# Autodesk Inventor assembly: erp42
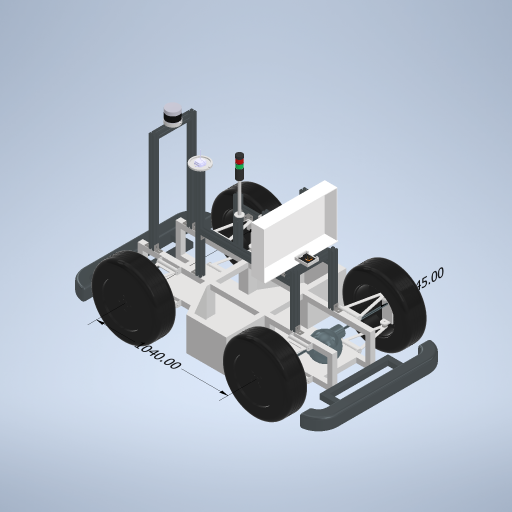
[picture p0: Inventor's stored thumbnail of the model, 512x512]
Saved by Autodesk Inventor 2023 (Build 270158000, 158)
## iProperties
Created: 2024-02-06
Part Number: erp42
Document SubType Name: Assembly
Designer: ps737
Author: ps737
## Documents named in this file (29)
- C:\Users\ps737\OneDrive\바탕 화면\2024 ERP42\erp42.iam
- C:\Users\ps737\OneDrive\바탕 화면\2024 ERP42\body.ipt
- C:\Users\ps737\OneDrive\바탕 화면\2024 ERP42\bumper.ipt
- C:\Users\ps737\OneDrive\바탕 화면\2024 ERP42\body_braket.ipt
- C:\Users\ps737\OneDrive\바탕 화면\2024 ERP42\link.ipt
- C:\Users\ps737\OneDrive\바탕 화면\2024 ERP42\wheel.ipt
- C:\Users\ps737\OneDrive\바탕 화면\2024 ERP42\wheel_bolt.ipt
- C:\Users\ps737\OneDrive\바탕 화면\2024 ERP42\프로파일\34.ipt
- C:\Users\ps737\OneDrive\바탕 화면\2024 ERP42\프로파일\76.ipt
- C:\Users\ps737\OneDrive\바탕 화면\2024 ERP42\프로파일\79.ipt
- C:\Users\ps737\OneDrive\바탕 화면\2024 ERP42\프로파일\26.ipt
- C:\Users\ps737\OneDrive\바탕 화면\2024 ERP42\프로파일\71.ipt
- C:\Users\ps737\OneDrive\바탕 화면\2024 ERP42\lidar_case.ipt
- C:\Users\ps737\OneDrive\바탕 화면\2024 ERP42\86-0138 REV 2, ENVELOPE, VLP-32C M12M.iam
- C:\Users\ps737\OneDrive\바탕 화면\2024 ERP42\gps_case.ipt
- C:\Users\ps737\OneDrive\바탕 화면\2024 ERP42\UBLOX_ANN-MB-00_GNSS_ANTENNA.ipt
- C:\Users\ps737\OneDrive\바탕 화면\2024 ERP42\프로파일\40.5.ipt
- C:\Users\ps737\OneDrive\바탕 화면\2024 ERP42\imu_case.ipt
- C:\Users\ps737\OneDrive\바탕 화면\2024 ERP42\MTi 600-series STEP files\MTi-600 DEV assembly.iam
- C:\Users\ps737\OneDrive\바탕 화면\2024 ERP42\L자 브라켓.ipt
- C:\Users\ps737\OneDrive\바탕 화면\2024 ERP42\wheel_braket_13.ipt
- C:\Users\ps737\OneDrive\바탕 화면\2024 ERP42\wheel_braket_24.ipt
- C:\Users\ps737\OneDrive\바탕 화면\2024 ERP42\base_link.ipt
- base_link.ipt
- C:\Users\ps737\OneDrive\바탕 화면\2024 ERP42\gps_case_2.ipt
- C:\Users\ps737\OneDrive\바탕 화면\2024 ERP42\프로파일\8.ipt
- C:\Users\ps737\OneDrive\바탕 화면\2024 ERP42\프로파일\36.ipt
- C:\Users\ps737\OneDrive\바탕 화면\2024 ERP42\monitor_case.ipt
- C:\Users\ps737\OneDrive\바탕 화면\2024 ERP42\led.ipt
## Components (74 placed, 27 different names)
1. body:1 — 메이트:1, 메이트:2, 메이트:3, 메이트:4, 메이트:5, 메이트:6, 메이트:9, 메이트:12, 메이트:60, 메이트:61, 플러쉬:1, 플러쉬:3, 플러쉬:4, 메이트:62, 메이트:64, 메이트:65, 플러쉬:6, 플러쉬:7, 플러쉬:8, 메이트:77, 메이트:78, 메이트:79, 플러쉬:9, 플러쉬:10, 플러쉬:11, 메이트:86, 메이트:89, 플러쉬:16, 메이트:90, 메이트:91, 플러쉬:17, 플러쉬:18, 메이트:107, 메이트:108, 플러쉬:21, 플러쉬:22, 메이트:109, 메이트:110, 메이트:124, 플러쉬:28, 각도:18, 플러쉬:29, 각도:19, 플러쉬:31, 플러쉬:32, 플러쉬:33, 메이트:152, 메이트:153, 메이트:154, 각도:20, 각도:21, 각도:22, 각도:23, 메이트:192, 플러쉬:34, 메이트:194, 플러쉬:35, 메이트:196, 플러쉬:36, 메이트:198, 플러쉬:37, 메이트:200, 플러쉬:38, 메이트:202, 플러쉬:39, 메이트:204, 메이트:206, 플러쉬:41, 메이트:209, 플러쉬:42, 메이트:241, 메이트:242
2. bumper:1 — 메이트:1, 메이트:2, 플러쉬:6, 플러쉬:10
3. bumper:2 — 메이트:3, 메이트:4, 플러쉬:7, 플러쉬:11, 플러쉬:58
4. body_braket:5 — 메이트:5, 플러쉬:32, 메이트:145, 메이트:151, 메이트:153
5. body_braket:7 — 메이트:6, 메이트:133, 메이트:134, 플러쉬:29, 플러쉬:30
6. body_braket:10 — 메이트:9, 플러쉬:3, 메이트:65, 메이트:144, 메이트:150
7. body_braket:12 — 메이트:12, 플러쉬:1, 메이트:62, 메이트:135, 메이트:136, 플러쉬:30, 플러쉬:40
8. body_braket:15 — 메이트:61, 메이트:140, 메이트:143, 플러쉬:31, 메이트:154
9. body_braket:16 — 메이트:60, 플러쉬:4, 메이트:64, 메이트:141, 메이트:142
10. body_braket:17 — 메이트:79, 플러쉬:33, 메이트:146, 메이트:148, 메이트:152
11. body_braket:18 — 메이트:77, 메이트:78, 플러쉬:9, 메이트:147, 메이트:149
12. 76:1 — 메이트:86, 메이트:89, 플러쉬:16, 메이트:105, 메이트:106, 각도:15, 각도:16, 메이트:207, 메이트:229, 플러쉬:54, 메이트:233
13. 79:1 — 메이트:90, 플러쉬:18, 메이트:94, 플러쉬:19, 플러쉬:20, 메이트:122, 메이트:193, 메이트:195
14. 79:2 — 메이트:91, 플러쉬:17, 메이트:123, 메이트:197, 메이트:199
15. 26:1 — 메이트:94, 플러쉬:19, 플러쉬:20, 메이트:101, 각도:13, 메이트:102
16. lidar_case:1 — 메이트:99, 메이트:100, 각도:12, 메이트:101
17. 86-0138 REV 2, ENVELOPE, VLP-32C M12M:1 [sub-assembly] — 메이트:99, 메이트:100, 각도:12, 각도:13, 메이트:102
18. gps_case:1 — 메이트:103, 각도:14, 메이트:104, 메이트:105, 메이트:106, 각도:16
19. UBLOX_ANN-MB-00_GNSS_ANTENNA:1 — 메이트:103, 각도:14, 메이트:104, 각도:15
20. 40.5:1 — 메이트:107, 플러쉬:21, 메이트:109, 메이트:111, 플러쉬:23, 플러쉬:24, 플러쉬:25, 메이트:201, 메이트:225, 플러쉬:52, 플러쉬:59
21. 40.5:2 — 메이트:108, 플러쉬:22, 메이트:110, 메이트:112, 메이트:114, 플러쉬:26, 메이트:205, 플러쉬:42, 메이트:224, 플러쉬:51
22. 34:1 — 메이트:111, 플러쉬:23, 플러쉬:24, 메이트:113, 메이트:115, 메이트:119, 메이트:120, 각도:17, 메이트:122, 메이트:123, 메이트:220, 메이트:222
23. 71:1 — 메이트:112, 메이트:113, 플러쉬:25, 메이트:211, 메이트:221, 플러쉬:48, 메이트:226, 메이트:230, 메이트:231, 플러쉬:55, 메이트:235, 플러쉬:57
24. 71:2 — 메이트:114, 플러쉬:26, 메이트:115, 메이트:125, 플러쉬:43, 메이트:213, 플러쉬:44, 메이트:215, 메이트:216, 플러쉬:46, 메이트:219, 플러쉬:49, 플러쉬:50, 메이트:223, 메이트:228, 메이트:232, 플러쉬:56
25. imu_case:1 — 메이트:116, 메이트:117, 메이트:118, 메이트:119, 메이트:120, 각도:17
26. MTi-600 DEV assembly:1 [sub-assembly] — 메이트:116, 메이트:117, 메이트:118
27. 40.5:3 — 메이트:124, 플러쉬:28, 메이트:125, 메이트:203, 메이트:212, 메이트:214, 메이트:227, 플러쉬:53, 메이트:234
28. link:19 — 메이트:129, 메이트:130, 메이트:133, 메이트:134
29. wheel_braket_13:1 — 메이트:131, 메이트:132, 각도:19, 메이트:137, 메이트:139, 메이트:179, 각도:23, 메이트:185
30. wheel_bolt:11 — 메이트:129, 메이트:130, 메이트:131, 메이트:132
31. link:20 — 메이트:135, 메이트:136, 각도:18, 메이트:138, 메이트:240
32. wheel_bolt:12 — 메이트:137, 메이트:138, 메이트:139, 메이트:240
33. link:21 — 메이트:141, 메이트:142, 메이트:175, 메이트:177
34. link:22 — 메이트:140, 메이트:143, 메이트:176, 메이트:178, 메이트:184
35. link:23 — 메이트:146, 메이트:148, 메이트:172, 메이트:174
36. link:24 — 메이트:147, 메이트:149, 메이트:171, 메이트:173
37. link:25 — 메이트:144, 메이트:150, 메이트:167, 메이트:168
38. link:26 — 메이트:145, 메이트:151, 메이트:169, 메이트:170
39. wheel:1 — 메이트:186, 메이트:187
40. wheel:2 — 메이트:179, 메이트:185
41. wheel:3 — 메이트:190, 메이트:191
42. wheel:4 — 메이트:188, 메이트:189, 메이트:208, 메이트:210
43. wheel_braket_13:2 — 메이트:155, 메이트:156, 메이트:161, 메이트:162, 각도:21, 메이트:190, 메이트:191
44. wheel_braket_24:1 — 메이트:180, 메이트:181, 메이트:182, 메이트:183, 각도:20, 메이트:186, 메이트:187
45. wheel_braket_24:2 — 메이트:157, 메이트:158, 메이트:163, 메이트:164, 각도:22, 메이트:188, 메이트:189
46. wheel_bolt:13 — 메이트:158, 메이트:163, 메이트:172, 메이트:174
47. wheel_bolt:14 — 메이트:155, 메이트:161, 메이트:169, 메이트:170
48. wheel_bolt:15 — 메이트:157, 메이트:164, 메이트:171, 메이트:173
49. wheel_bolt:16 — 메이트:156, 메이트:162, 메이트:167, 메이트:168
50. wheel_bolt:17 — 메이트:175, 메이트:177, 메이트:180, 메이트:181, 메이트:183
51. wheel_bolt:18 — 메이트:176, 메이트:178, 메이트:182, 메이트:184
52. L자 브라켓:1 — 메이트:194, 메이트:195, 플러쉬:35
53. L자 브라켓:2 — 메이트:192, 메이트:193, 플러쉬:34
54. L자 브라켓:3 — 메이트:196, 메이트:197, 플러쉬:36
55. L자 브라켓:4 — 메이트:198, 메이트:199, 플러쉬:37
56. L자 브라켓:5 — 메이트:202, 메이트:203, 플러쉬:39
57. L자 브라켓:6 — 메이트:200, 메이트:201, 플러쉬:38, 플러쉬:59
58. L자 브라켓:7 — 메이트:204, 메이트:205, 플러쉬:40
59. L자 브라켓:8 — 메이트:206, 메이트:207, 플러쉬:41
60. base_link:1 — 메이트:208, 메이트:209, 메이트:210
61. gps_case_2:1 — 메이트:211, 메이트:212, 플러쉬:43
62. 8:1 — 메이트:213, 플러쉬:44, 메이트:214, 메이트:217, 메이트:218, 메이트:237, 메이트:238, 메이트:239
63. L자 브라켓:9 — 메이트:215, 플러쉬:46, 메이트:217
64. L자 브라켓:10 — 메이트:216, 메이트:218, 플러쉬:50
65. L자 브라켓:11 — 메이트:219, 메이트:220, 플러쉬:49
66. L자 브라켓:12 — 메이트:221, 메이트:222, 플러쉬:48
67. L자 브라켓:13 — 메이트:229, 메이트:230, 플러쉬:54
68. L자 브라켓:14 — 메이트:223, 메이트:224, 플러쉬:51
69. L자 브라켓:15 — 메이트:225, 메이트:226, 플러쉬:52
70. L자 브라켓:17 — 메이트:227, 메이트:228, 플러쉬:53
71. 36:1 — 메이트:231, 플러쉬:55, 메이트:233, 메이트:236
72. 36:2 — 메이트:232, 플러쉬:56, 메이트:234
73. monitor_case:1 — 메이트:235, 메이트:236, 플러쉬:57
74. led:1 — 메이트:237, 메이트:238, 메이트:239
## Relationships (219: Mate 157, Flush 50, Angle 12)
- 메이트:1 [Mate]: body:1 ↔ bumper:1
- 메이트:2 [Mate]: body:1 ↔ bumper:1
- 메이트:3 [Mate]: body:1 ↔ bumper:2
- 메이트:4 [Mate]: body:1 ↔ bumper:2
- 메이트:5 [Mate]: body:1 ↔ body_braket:5
- 메이트:6 [Mate]: body:1 ↔ body_braket:7
- 메이트:9 [Mate]: body:1 ↔ body_braket:10
- 메이트:12 [Mate]: body:1 ↔ body_braket:12
- 메이트:60 [Mate]: body:1 ↔ body_braket:16
- 메이트:61 [Mate]: body:1 ↔ body_braket:15
- 플러쉬:1 [Flush]: body:1 ↔ body_braket:12
- 플러쉬:3 [Flush]: body:1 ↔ body_braket:10
- 플러쉬:4 [Flush]: body:1 ↔ body_braket:16
- 메이트:62 [Mate] (230 mm): body:1 ↔ body_braket:12
- 메이트:64 [Mate] (190 mm): body:1 ↔ body_braket:16
- 메이트:65 [Mate] (190 mm): body:1 ↔ body_braket:10
- 플러쉬:6 [Flush] (-25 mm): body:1 ↔ bumper:1
- 플러쉬:7 [Flush] (-25 mm): body:1 ↔ bumper:2
- 플러쉬:8 [Flush] (105 mm): body:1
- 메이트:77 [Mate]: body:1 ↔ body_braket:18
- 메이트:78 [Mate] (230 mm): body:1 ↔ body_braket:18
- 메이트:79 [Mate]: body:1 ↔ body_braket:17
- 플러쉬:9 [Flush]: body:1 ↔ body_braket:18
- 플러쉬:10 [Flush] (100 mm): body:1 ↔ bumper:1
- 플러쉬:11 [Flush] (100 mm): body:1 ↔ bumper:2
- 메이트:86 [Mate]: body:1 ↔ 76:1
- 메이트:89 [Mate] (40 mm): body:1 ↔ 76:1
- 플러쉬:16 [Flush]: body:1 ↔ 76:1
- 메이트:90 [Mate]: body:1 ↔ 79:1
- 메이트:91 [Mate]: body:1 ↔ 79:2
- 플러쉬:17 [Flush]: body:1 ↔ 79:2
- 플러쉬:18 [Flush]: body:1 ↔ 79:1
- 메이트:94 [Mate]: 79:1 ↔ 26:1
- 플러쉬:19 [Flush]: 79:1 ↔ 26:1
- 플러쉬:20 [Flush]: 79:1 ↔ 26:1
- 메이트:99 [Mate]: lidar_case:1 ↔ 86-0138 REV 2, ENVELOPE, VLP-32C M12M:1
- 메이트:100 [Mate]: lidar_case:1 ↔ 86-0138 REV 2, ENVELOPE, VLP-32C M12M:1
- 각도:12 [Angle] (270 deg): lidar_case:1 ↔ 86-0138 REV 2, ENVELOPE, VLP-32C M12M:1
- 메이트:101 [Mate]: 26:1 ↔ lidar_case:1
- 각도:13 [Angle] (0 deg): 26:1 ↔ 86-0138 REV 2, ENVELOPE, VLP-32C M12M:1
- 메이트:102 [Mate]: 26:1 ↔ 86-0138 REV 2, ENVELOPE, VLP-32C M12M:1
- 메이트:103 [Mate]: gps_case:1 ↔ UBLOX_ANN-MB-00_GNSS_ANTENNA:1
- 각도:14 [Angle] (270 deg): gps_case:1 ↔ UBLOX_ANN-MB-00_GNSS_ANTENNA:1
- 메이트:104 [Mate]: gps_case:1 ↔ UBLOX_ANN-MB-00_GNSS_ANTENNA:1
- 메이트:105 [Mate]: 76:1 ↔ gps_case:1
- 메이트:106 [Mate]: 76:1 ↔ gps_case:1
- 각도:15 [Angle] (0 deg): 76:1 ↔ UBLOX_ANN-MB-00_GNSS_ANTENNA:1
- 각도:16 [Angle] (270 deg): 76:1 ↔ gps_case:1
- 메이트:107 [Mate]: body:1 ↔ 40.5:1
- 메이트:108 [Mate]: body:1 ↔ 40.5:2
- 플러쉬:21 [Flush]: body:1 ↔ 40.5:1
- 플러쉬:22 [Flush]: body:1 ↔ 40.5:2
- 메이트:109 [Mate] (200 mm): body:1 ↔ 40.5:1
- 메이트:110 [Mate] (200 mm): body:1 ↔ 40.5:2
- 메이트:111 [Mate]: 40.5:1 ↔ 34:1
- 플러쉬:23 [Flush]: 40.5:1 ↔ 34:1
- 플러쉬:24 [Flush] (28 mm): 40.5:1 ↔ 34:1
- 메이트:112 [Mate]: 40.5:2 ↔ 71:1
- 메이트:113 [Mate]: 34:1 ↔ 71:1
- 플러쉬:25 [Flush]: 40.5:1 ↔ 71:1
- 메이트:114 [Mate]: 40.5:2 ↔ 71:2
- 플러쉬:26 [Flush]: 40.5:2 ↔ 71:2
- 메이트:115 [Mate]: 34:1 ↔ 71:2
- 메이트:116 [Mate]: imu_case:1 ↔ MTi-600 DEV assembly:1
- 메이트:117 [Mate]: imu_case:1 ↔ MTi-600 DEV assembly:1
- 메이트:118 [Mate]: imu_case:1 ↔ MTi-600 DEV assembly:1
- 메이트:119 [Mate]: 34:1 ↔ imu_case:1
- 메이트:120 [Mate]: 34:1 ↔ imu_case:1
- 각도:17 [Angle] (0 deg): 34:1 ↔ imu_case:1
- 메이트:122 [Mate] (1038 mm): 79:1 ↔ 34:1
- 메이트:123 [Mate] (1038 mm): 79:2 ↔ 34:1
- 메이트:124 [Mate]: body:1 ↔ 40.5:3
- 플러쉬:28 [Flush]: body:1 ↔ 40.5:3
- 메이트:125 [Mate]: 71:2 ↔ 40.5:3
- 메이트:129 [Mate]: link:19 ↔ wheel_bolt:11
- 메이트:130 [Mate]: link:19 ↔ wheel_bolt:11
- 메이트:131 [Mate]: wheel_braket_13:1 ↔ wheel_bolt:11
- 메이트:132 [Mate]: wheel_braket_13:1 ↔ wheel_bolt:11
- 메이트:133 [Mate]: body_braket:7 ↔ link:19
- 메이트:134 [Mate]: body_braket:7 ↔ link:19
- 메이트:135 [Mate]: body_braket:12 ↔ link:20
- 메이트:136 [Mate]: body_braket:12 ↔ link:20
- 각도:18 [Angle] (0 deg): body:1 ↔ link:20
- 플러쉬:29 [Flush]: body:1 ↔ body_braket:7
- 각도:19 [Angle] (180 deg): body:1 ↔ wheel_braket_13:1
- 플러쉬:30 [Flush]: body_braket:7 ↔ body_braket:12
- 메이트:137 [Mate]: wheel_braket_13:1 ↔ wheel_bolt:12
- 메이트:138 [Mate]: link:20 ↔ wheel_bolt:12
- 메이트:139 [Mate]: wheel_braket_13:1 ↔ wheel_bolt:12
- 메이트:140 [Mate]: body_braket:15 ↔ link:22
- 메이트:141 [Mate]: body_braket:16 ↔ link:21
- 메이트:142 [Mate]: body_braket:16 ↔ link:21
- 메이트:143 [Mate]: body_braket:15 ↔ link:22
- 플러쉬:31 [Flush]: body:1 ↔ body_braket:15
- 플러쉬:32 [Flush]: body:1 ↔ body_braket:5
- 플러쉬:33 [Flush]: body:1 ↔ body_braket:17
- 메이트:144 [Mate]: body_braket:10 ↔ link:25
- 메이트:145 [Mate]: body_braket:5 ↔ link:26
- 메이트:146 [Mate]: body_braket:17 ↔ link:23
- 메이트:147 [Mate]: body_braket:18 ↔ link:24
- 메이트:148 [Mate]: body_braket:17 ↔ link:23
- 메이트:149 [Mate]: body_braket:18 ↔ link:24
- 메이트:150 [Mate]: body_braket:10 ↔ link:25
- 메이트:151 [Mate]: body_braket:5 ↔ link:26
- 메이트:152 [Mate] (230 mm): body:1 ↔ body_braket:17
- 메이트:153 [Mate] (190 mm): body:1 ↔ body_braket:5
- 메이트:154 [Mate] (190 mm): body:1 ↔ body_braket:15
- 메이트:155 [Mate]: wheel_braket_13:2 ↔ wheel_bolt:14
- 메이트:156 [Mate]: wheel_braket_13:2 ↔ wheel_bolt:16
- 메이트:157 [Mate]: wheel_braket_24:2 ↔ wheel_bolt:15
- 메이트:158 [Mate]: wheel_braket_24:2 ↔ wheel_bolt:13
- 메이트:161 [Mate]: wheel_braket_13:2 ↔ wheel_bolt:14
- 메이트:162 [Mate]: wheel_braket_13:2 ↔ wheel_bolt:16
- 메이트:163 [Mate]: wheel_braket_24:2 ↔ wheel_bolt:13
- 메이트:164 [Mate]: wheel_braket_24:2 ↔ wheel_bolt:15
- 메이트:167 [Mate]: link:25 ↔ wheel_bolt:16
- 메이트:168 [Mate]: link:25 ↔ wheel_bolt:16
- 메이트:169 [Mate]: link:26 ↔ wheel_bolt:14
- 메이트:170 [Mate]: link:26 ↔ wheel_bolt:14
- 메이트:171 [Mate]: link:24 ↔ wheel_bolt:15
- 메이트:172 [Mate]: link:23 ↔ wheel_bolt:13
- 메이트:173 [Mate]: link:24 ↔ wheel_bolt:15
- 메이트:174 [Mate]: link:23 ↔ wheel_bolt:13
- 메이트:175 [Mate]: link:21 ↔ wheel_bolt:17
- 메이트:176 [Mate]: link:22 ↔ wheel_bolt:18
- 메이트:177 [Mate]: link:21 ↔ wheel_bolt:17
- 메이트:178 [Mate]: link:22 ↔ wheel_bolt:18
- 메이트:179 [Mate]: wheel_braket_13:1 ↔ wheel:2
- 메이트:180 [Mate]: wheel_braket_24:1 ↔ wheel_bolt:17
- 메이트:181 [Mate]: wheel_braket_24:1 ↔ wheel_bolt:17
- 메이트:182 [Mate]: wheel_braket_24:1 ↔ wheel_bolt:18
- 메이트:183 [Mate]: wheel_braket_24:1 ↔ wheel_bolt:17
- 메이트:184 [Mate]: link:22 ↔ wheel_bolt:18
- 각도:20 [Angle] (180 deg): body:1 ↔ wheel_braket_24:1
- 각도:21 [Angle] (180 deg): body:1 ↔ wheel_braket_13:2
- 각도:22 [Angle] (180 deg): body:1 ↔ wheel_braket_24:2
- 각도:23 [Angle] (180 deg): body:1 ↔ wheel_braket_13:1
- 메이트:185 [Mate]: wheel_braket_13:1 ↔ wheel:2
- 메이트:186 [Mate]: wheel:1 ↔ wheel_braket_24:1
- 메이트:187 [Mate]: wheel:1 ↔ wheel_braket_24:1
- 메이트:188 [Mate]: wheel:4 ↔ wheel_braket_24:2
- 메이트:189 [Mate]: wheel:4 ↔ wheel_braket_24:2
- 메이트:190 [Mate]: wheel:3 ↔ wheel_braket_13:2
- 메이트:191 [Mate]: wheel:3 ↔ wheel_braket_13:2
- 메이트:192 [Mate]: body:1 ↔ L자 브라켓:2
- 메이트:193 [Mate]: 79:1 ↔ L자 브라켓:2
- 플러쉬:34 [Flush] (2.5 mm): body:1 ↔ L자 브라켓:2
- 메이트:194 [Mate]: body:1 ↔ L자 브라켓:1
- 메이트:195 [Mate]: 79:1 ↔ L자 브라켓:1
- 플러쉬:35 [Flush] (2.5 mm): body:1 ↔ L자 브라켓:1
- 메이트:196 [Mate]: body:1 ↔ L자 브라켓:3
- 메이트:197 [Mate]: 79:2 ↔ L자 브라켓:3
- 플러쉬:36 [Flush] (2.2 mm): body:1 ↔ L자 브라켓:3
- 메이트:198 [Mate]: body:1 ↔ L자 브라켓:4
- 메이트:199 [Mate]: 79:2 ↔ L자 브라켓:4
- 플러쉬:37 [Flush] (2.5 mm): body:1 ↔ L자 브라켓:4
- 메이트:200 [Mate]: body:1 ↔ L자 브라켓:6
- 메이트:201 [Mate]: 40.5:1 ↔ L자 브라켓:6
- 플러쉬:38 [Flush] (2.5 mm): body:1 ↔ L자 브라켓:6
- 메이트:202 [Mate]: body:1 ↔ L자 브라켓:5
- 메이트:203 [Mate]: 40.5:3 ↔ L자 브라켓:5
- 플러쉬:39 [Flush] (2.5 mm): body:1 ↔ L자 브라켓:5
- 메이트:204 [Mate]: body:1 ↔ L자 브라켓:7
- 메이트:205 [Mate]: 40.5:2 ↔ L자 브라켓:7
- 플러쉬:40 [Flush] (2.5 mm): body_braket:12 ↔ L자 브라켓:7
- 메이트:206 [Mate]: body:1 ↔ L자 브라켓:8
- 메이트:207 [Mate]: 76:1 ↔ L자 브라켓:8
- 플러쉬:41 [Flush] (2.5 mm): body:1 ↔ L자 브라켓:8
- 메이트:208 [Mate]: wheel:4 ↔ base_link:1
- 메이트:209 [Mate]: body:1 ↔ base_link:1
- 메이트:210 [Mate]: wheel:4 ↔ base_link:1
- 메이트:211 [Mate]: 71:1 ↔ gps_case_2:1
- 플러쉬:42 [Flush]: body:1 ↔ 40.5:2
- 메이트:212 [Mate] (170 mm): 40.5:3 ↔ gps_case_2:1
- 플러쉬:43 [Flush] (12.5 mm): 71:2 ↔ gps_case_2:1
- 메이트:213 [Mate]: 71:2 ↔ 8:1
- 플러쉬:44 [Flush]: 71:2 ↔ 8:1
- 메이트:214 [Mate] (40 mm): 40.5:3 ↔ 8:1
- 메이트:215 [Mate]: 71:2 ↔ L자 브라켓:9
- 메이트:216 [Mate]: 71:2 ↔ L자 브라켓:10
- 플러쉬:46 [Flush] (2.5 mm): 71:2 ↔ L자 브라켓:9
- 메이트:217 [Mate]: 8:1 ↔ L자 브라켓:9
- 메이트:218 [Mate]: 8:1 ↔ L자 브라켓:10
- 메이트:219 [Mate]: 71:2 ↔ L자 브라켓:11
- 메이트:220 [Mate]: 34:1 ↔ L자 브라켓:11
- 메이트:221 [Mate]: 71:1 ↔ L자 브라켓:12
- 메이트:222 [Mate]: 34:1 ↔ L자 브라켓:12
- 플러쉬:48 [Flush] (2.5 mm): 71:1 ↔ L자 브라켓:12
- 플러쉬:49 [Flush] (2.5 mm): 71:2 ↔ L자 브라켓:11
- 플러쉬:50 [Flush] (2.5 mm): 71:2 ↔ L자 브라켓:10
- 메이트:223 [Mate]: 71:2 ↔ L자 브라켓:14
- 메이트:224 [Mate]: 40.5:2 ↔ L자 브라켓:14
- 플러쉬:51 [Flush] (2.5 mm): 40.5:2 ↔ L자 브라켓:14
- 메이트:225 [Mate]: 40.5:1 ↔ L자 브라켓:15
- 메이트:226 [Mate]: 71:1 ↔ L자 브라켓:15
- 플러쉬:52 [Flush] (2.5 mm): 40.5:1 ↔ L자 브라켓:15
- 메이트:227 [Mate]: 40.5:3 ↔ L자 브라켓:17
- 메이트:228 [Mate]: 71:2 ↔ L자 브라켓:17
- 플러쉬:53 [Flush] (2.5 mm): 40.5:3 ↔ L자 브라켓:17
- 메이트:229 [Mate]: 76:1 ↔ L자 브라켓:13
- 메이트:230 [Mate]: 71:1 ↔ L자 브라켓:13
- 플러쉬:54 [Flush] (2.5 mm): 76:1 ↔ L자 브라켓:13
- 메이트:231 [Mate]: 71:1 ↔ 36:1
- 메이트:232 [Mate]: 71:2 ↔ 36:2
- 플러쉬:55 [Flush]: 71:1 ↔ 36:1
- 플러쉬:56 [Flush]: 71:2 ↔ 36:2
- 메이트:233 [Mate] (485 mm): 76:1 ↔ 36:1
- 메이트:234 [Mate] (485 mm): 40.5:3 ↔ 36:2
- 메이트:235 [Mate]: 71:1 ↔ monitor_case:1
- 메이트:236 [Mate]: 36:1 ↔ monitor_case:1
- 플러쉬:57 [Flush] (-120 mm): 71:1 ↔ monitor_case:1
- 메이트:237 [Mate]: 8:1 ↔ led:1
- 메이트:238 [Mate] (10 mm): 8:1 ↔ led:1
- 메이트:239 [Mate] (20 mm): 8:1 ↔ led:1
- 메이트:240 [Mate]: link:20 ↔ wheel_bolt:12
- 메이트:241 [Mate] (-170 mm): body:1
- 메이트:242 [Mate] (105 mm): body:1
- 플러쉬:58 [Flush] (-990 mm): bumper:2
- 플러쉬:59 [Flush] (2.5 mm): 40.5:1 ↔ L자 브라켓:6
